# Autodesk Inventor assembly: cw12model
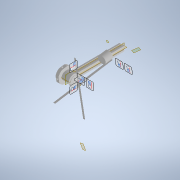
[picture p0: Inventor's stored thumbnail of the model, 180x180]
Saved by Autodesk Inventor 2021 (Build 250183000, 183)
## iProperties
Created: 2021-06-18
Part Number: cw12model
Document SubType Name: Assembly
Designer: Wojciech Wołczek
Author: Wojciech Wołczek
## Documents named in this file (6)
- D:\OneDrive\Documents\studia\I rok\labolatoria pracowni fizycznej\pracownia fizyczna 2021 xD\cw 12\cw12model.iam
- D:\OneDrive\Documents\studia\I rok\labolatoria pracowni fizycznej\pracownia fizyczna 2021 xD\cw 2\wysiegnik.ipt
- D:\OneDrive\Documents\studia\I rok\labolatoria pracowni fizycznej\pracownia fizyczna 2021 xD\cw 2\jakis_modulxD.ipt
- D:\OneDrive\Documents\studia\I rok\labolatoria pracowni fizycznej\pracownia fizyczna 2021 xD\cw 2\shaft.ipt
- D:\OneDrive\Documents\studia\I rok\labolatoria pracowni fizycznej\pracownia fizyczna 2021 xD\cw 12\rurka.ipt
- D:\OneDrive\Documents\studia\I rok\labolatoria pracowni fizycznej\pracownia fizyczna 2021 xD\cw 12\ciezarek1.ipt
## Components (6 placed, 5 different names)
1. wysiegnik:1 — Równoległe:1, Zestawiające:1, Równoległe:15, Zestawiające:2, Zestawiające:3
2. jakis_modulxD:1 — Równoległe:1, Równoległe:3, Zestawiające:1, Zestawiające:2, Zestawiające:3
3. shaft:1 — Równoległe:3, Równoległe:4, Równoległe:5
4. ciezarek1:1 — Równoległe:6, Równoległe:7
5. rurka:1 — Równoległe:4, Równoległe:5
6. rurka:2 — Równoległe:6, Równoległe:7
## Component patterns: (2 elements, first: rurka:1)
## Relationships (10: Flush 7, Mate 3)
- Równoległe:1 [Flush]: wysiegnik:1 ↔ jakis_modulxD:1
- Równoległe:3 [Flush]: jakis_modulxD:1 ↔ shaft:1
- Równoległe:4 [Flush]: shaft:1 ↔ rurka:1
- Równoległe:5 [Flush]: shaft:1 ↔ rurka:1
- Równoległe:6 [Flush]: ciezarek1:1 ↔ rurka:2
- Równoległe:7 [Flush] (-25 mm): ciezarek1:1 ↔ rurka:2
- Zestawiające:1 [Mate]: wysiegnik:1 ↔ jakis_modulxD:1
- Równoległe:15 [Flush]: wysiegnik:1
- Zestawiające:2 [Mate]: wysiegnik:1 ↔ jakis_modulxD:1
- Zestawiające:3 [Mate]: wysiegnik:1 ↔ jakis_modulxD:1
